# Autodesk Inventor assembly: neck_link
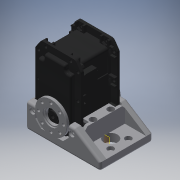
[picture p0: Inventor's stored thumbnail of the model, 180x180]
Saved by Autodesk Inventor 2018 (Build 220112000, 112)
## iProperties
Created: 2018-12-01
Part Number: neck_link
Document SubType Name: Assembly
Designer: jaspe
Author: jaspe
## Documents named in this file (3)
- C:\Users\jaspe\bitbots_hardware\wolfgang\assembly\head\neck_link.iam
- C:\Users\jaspe\bitbots_hardware\wolfgang\assembly\head\hals.ipt
- C:\Users\jaspe\bitbots_hardware\wolfgang\assembly\motors\MX64\Mx64_with_bearing.iam
## Components (2 placed, 2 different names)
1. hals:1 — Mate:1, Mate:2, Mate:3, Mate:4, Mate:5, Mate:6
2. Mx64_with_bearing:1 [sub-assembly] — Mate:4, Mate:5, Mate:6
## Relationships (6: Mate 6)
- Mate:1: hals:1
- Mate:2: hals:1
- Mate:3: hals:1
- Mate:4: hals:1 ↔ Mx64_with_bearing:1
- Mate:5: hals:1 ↔ Mx64_with_bearing:1
- Mate:6: hals:1 ↔ Mx64_with_bearing:1
